# Autodesk Inventor assembly: Bumper Half Assembly
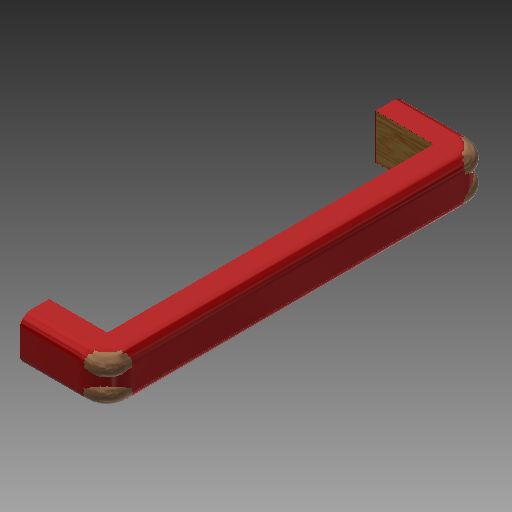
[picture p0: Inventor's stored thumbnail of the model, 512x512]
Saved by Autodesk Inventor 2019.4 (Build 234330000, 330)
## iProperties
Created: 2020-01-22
Part Number: Bumper Half Assembly
Document SubType Name: Assembly
Designer: admin
Author: admin
## Documents named in this file (5)
- C:\Users\Mark\Desktop\7738 Helion Engineering\7738-2020\Robot V2\Bumper\Bumper Half Assembly.iam
- C:\Users\Mark\Desktop\7738 Helion Engineering\7738-2020\Robot V2\Bumper\Bumper Wood 1.ipt
- C:\Users\Mark\Desktop\7738 Helion Engineering\7738-2020\Robot V2\Bumper\Bumper Wood 2.ipt
- C:\Users\Mark\Desktop\7738 Helion Engineering\7738-2020\Robot V2\Bumper\Pool Noodle.ipt
- C:\Users\Mark\Desktop\7738 Helion Engineering\7738-2020\Robot V2\Bumper\Bumper Fabric.ipt
## Components (6 placed, 4 different names)
1. Bumper Wood 1:1 — Mate:1, Flush:1, Flush:2, Mate:2, Flush:3, Flush:4, Tangent:2, Tangent:3, Tangent:5
2. Bumper Wood 2:1 — Mate:1, Flush:1, Flush:2, Tangent:6, Angle:1
3. Bumper Wood 2:2 — Mate:2, Flush:3, Flush:4, Tangent:1, Flush:5, Tangent:4, Flush:6
4. Pool Noodle:1 — Tangent:4, Tangent:5, Flush:6, Tangent:6, Tangent:7
5. Pool Noodle:2 — Tangent:1, Tangent:2, Tangent:3, Flush:5, Tangent:7, Mate:4
6. Bumper Fabric:1 — Mate:4, Angle:1
## Relationships (17: Tangent 7, Flush 6, Mate 3, Angle 1)
- Mate:1: Bumper Wood 1:1 ↔ Bumper Wood 2:1
- Flush:1: Bumper Wood 1:1 ↔ Bumper Wood 2:1
- Flush:2: Bumper Wood 1:1 ↔ Bumper Wood 2:1
- Mate:2: Bumper Wood 1:1 ↔ Bumper Wood 2:2
- Flush:3: Bumper Wood 1:1 ↔ Bumper Wood 2:2
- Flush:4: Bumper Wood 1:1 ↔ Bumper Wood 2:2
- Tangent:1: Bumper Wood 2:2 ↔ Pool Noodle:2
- Tangent:2: Bumper Wood 1:1 ↔ Pool Noodle:2
- Tangent:3: Bumper Wood 1:1 ↔ Pool Noodle:2
- Flush:5: Bumper Wood 2:2 ↔ Pool Noodle:2
- Tangent:4: Bumper Wood 2:2 ↔ Pool Noodle:1
- Tangent:5: Bumper Wood 1:1 ↔ Pool Noodle:1
- Flush:6: Bumper Wood 2:2 ↔ Pool Noodle:1
- Tangent:6: Bumper Wood 2:1 ↔ Pool Noodle:1
- Tangent:7: Pool Noodle:1 ↔ Pool Noodle:2
- Mate:4: Pool Noodle:2 ↔ Bumper Fabric:1
- Angle:1 (0 deg): Bumper Wood 2:1 ↔ Bumper Fabric:1
